# Autodesk Inventor assembly: Assembly1
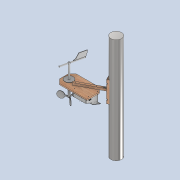
[picture p0: Inventor's stored thumbnail of the model, 180x180]
Saved by Autodesk Inventor 2022 (Build 260153000, 153)
## iProperties
Created: 2025-07-11
Part Number: Assembly1
Document SubType Name: Assembly
Designer: 1234
Author: 1234
## Documents named in this file (23)
- C:\Users\1234\Dropbox\Giorgio_Mac\PPS (pascon piccone sacchiero)\componenti\spot\IPT\Assembly1.iam
- C:\Users\1234\Dropbox\Giorgio_Mac\PPS (pascon piccone sacchiero)\componenti\spot\IPT\pannello solare.ipt
- C:\Users\1234\Dropbox\Giorgio_Mac\PPS (pascon piccone sacchiero)\componenti\spot\IPT\scatola - coperchio principale.ipt
- C:\Users\1234\Dropbox\Giorgio_Mac\PPS (pascon piccone sacchiero)\componenti\spot\IPT\Tower Pro MG996R.ipt
- C:\Users\1234\Dropbox\Giorgio_Mac\PPS (pascon piccone sacchiero)\componenti\spot\IPT\guarnizione motore.ipt
- C:\Users\1234\Dropbox\Giorgio_Mac\PPS (pascon piccone sacchiero)\componenti\spot\IPT\adattatore per motore.ipt
- C:\Users\1234\Dropbox\Giorgio_Mac\PPS (pascon piccone sacchiero)\componenti\spot\IPT\cupola alta di protezione.ipt
- C:\Users\1234\Dropbox\Giorgio_Mac\PPS (pascon piccone sacchiero)\componenti\spot\IPT\manometro.ipt
- C:\Users\1234\Dropbox\Giorgio_Mac\PPS (pascon piccone sacchiero)\componenti\spot\IPT\legno.ipt
- C:\Users\1234\Dropbox\Giorgio_Mac\PPS (pascon piccone sacchiero)\componenti\spot\IPT\direzione del vento.ipt
- C:\Users\1234\Dropbox\Giorgio_Mac\PPS (pascon piccone sacchiero)\componenti\spot\IPT\legno 1.ipt
- C:\Users\1234\Dropbox\Giorgio_Mac\PPS (pascon piccone sacchiero)\componenti\spot\IPT\legno 2.ipt
- C:\Users\1234\Dropbox\Giorgio_Mac\PPS (pascon piccone sacchiero)\componenti\spot\IPT\profiletto a l.ipt
- C:\Users\1234\Dropbox\Giorgio_Mac\PPS (pascon piccone sacchiero)\componenti\spot\IPT\lampione.ipt
- C:\Users\1234\Dropbox\Giorgio_Mac\PPS (pascon piccone sacchiero)\componenti\spot\IPT\spazzola - asta.ipt
- C:\Users\1234\Dropbox\Giorgio_Mac\PPS (pascon piccone sacchiero)\componenti\spot\IPT\spazzola - spazzola.ipt
- C:\Users\1234\Dropbox\Giorgio_Mac\PPS (pascon piccone sacchiero)\componenti\spot\IPT\spessori.ipt
- C:\Users\1234\Dropbox\Giorgio_Mac\PPS (pascon piccone sacchiero)\componenti\spot\IPT\piedino.ipt
- C:\Users\1234\Dropbox\Giorgio_Mac\PPS (pascon piccone sacchiero)\componenti\spot\IPT\tappino tpu.ipt
- C:\Users\1234\Dropbox\Giorgio_Mac\PPS (pascon piccone sacchiero)\componenti\spot\IPT\scatola - corpo - v2.ipt
- C:\Users\1234\Dropbox\Giorgio_Mac\PPS (pascon piccone sacchiero)\componenti\spot\IPT\spazzola - appoggio.ipt
- C:\Users\1234\Dropbox\Giorgio_Mac\PPS (pascon piccone sacchiero)\PCB\PCB_v2\3D_Sensor_Module_Rev_0_2025-09-11.iam
- C:\Users\1234\Dropbox\Giorgio_Mac\PPS (pascon piccone sacchiero)\componenti\spot\IPT\scatola - corpo - v3.ipt
## Components (28 placed, 22 different names)
1. scatola - coperchio principale:1 — Mate:47, Mate:49, Mate:86, Mate:109, Mate:110, Mate:134, Mate:138, Angle:3, Mate:139, Mate:145, Mate:146, Mate:147
2. pannello solare:2 — Mate:152, Angle:6
3. Tower Pro MG996R:1 — Mate:35, Mate:36, Mate:123, Mate:143, Mate:144
4. guarnizione motore:2 — Mate:125, Mate:126, Mate:127
5. adattatore per motore:2 — Mate:35, Mate:36, Mate:106, Mate:107, Mate:108
6. cupola alta di protezione:1 — Mate:140, Mate:141, Mate:142
7. legno:1 — Mate:47, Mate:49, Mate:50, Mate:54, Flush:1, Flush:2, Mate:55, Mate:56, Mate:57, Mate:64, Mate:66, Mate:78, Mate:79, Mate:80, Mate:81, Mate:82, Mate:83, Mate:84, Mate:85
8. manometro:1 — Mate:50, Mate:66, Mate:67
9. direzione del vento:1 — Mate:64, Mate:67
10. legno 1:1 — Mate:55, Mate:56, Mate:57, Mate:62, Mate:63, Flush:3, Flush:4, Mate:87, Mate:88
11. legno 2:1 — Mate:87, Mate:88, Mate:89, Mate:90, Angle:2, Mate:91
12. profiletto a l:1 — Mate:62, Flush:4, Mate:90
13. profiletto a l:2 — Mate:63, Flush:3, Mate:89
14. lampione:1 — Angle:1, Angle:2, Mate:91
15. spazzola - asta:1 — Mate:76, Flush:6, Mate:106, Mate:107, Mate:108, Mate:130
16. spazzola - spazzola:1 — Mate:76, Flush:6, Mate:130
17. spessori:1 — Mate:82, Mate:83
18. spessori:2 — Mate:81, Mate:84
19. spessori:3 — Mate:80, Mate:85, Mate:86
20. spessori:4 — Mate:78, Mate:79
21. piedino:3
22. tappino tpu:1 — Mate:148, Mate:149, Mate:150
23. scatola - corpo - v2:1 — Mate:109, Mate:110, Mate:113, Mate:123, Mate:125, Mate:126, Mate:127, Mate:131, Mate:132, Mate:134, Mate:140, Mate:141, Mate:142, Mate:143, Mate:144
24. spazzola - appoggio:1 — Mate:113, Mate:131, Mate:132
25. 3D_Sensor_Module_Rev_0_2025-09-11:1 [sub-assembly] — Mate:138, Angle:3, Mate:139
26. pannello solare:3 — Mate:151, Angle:4
27. scatola - corpo - v3:1 — Mate:145, Mate:146, Mate:147, Mate:148, Mate:149, Mate:150, Mate:151, Mate:152, Mate:153, Angle:4, Angle:5, Angle:6
28. pannello solare:4 — Mate:153, Angle:5
## Relationships (70: Mate 59, Angle 6, Flush 5)
- Mate:35: Tower Pro MG996R:1 ↔ adattatore per motore:2
- Mate:36 (0.5 mm): Tower Pro MG996R:1 ↔ adattatore per motore:2
- Mate:47: scatola - coperchio principale:1 ↔ legno:1
- Mate:49: scatola - coperchio principale:1 ↔ legno:1
- Mate:50: legno:1 ↔ manometro:1
- Mate:54: legno:1
- Flush:1: legno:1
- Flush:2: legno:1
- Mate:55: legno:1 ↔ legno 1:1
- Mate:56: legno:1 ↔ legno 1:1
- Mate:57: legno:1 ↔ legno 1:1
- Mate:62: legno 1:1 ↔ profiletto a l:1
- Mate:63: legno 1:1 ↔ profiletto a l:2
- Flush:3 (5 mm): legno 1:1 ↔ profiletto a l:2
- Flush:4 (5 mm): legno 1:1 ↔ profiletto a l:1
- Mate:64: legno:1 ↔ direzione del vento:1
- Mate:66: legno:1 ↔ manometro:1
- Mate:67: manometro:1 ↔ direzione del vento:1
- Mate:76 (0.1 mm): spazzola - asta:1 ↔ spazzola - spazzola:1
- Flush:6: spazzola - asta:1 ↔ spazzola - spazzola:1
- Mate:78: legno:1 ↔ spessori:4
- Mate:79: legno:1 ↔ spessori:4
- Mate:80: legno:1 ↔ spessori:3
- Mate:81: legno:1 ↔ spessori:2
- Mate:82: legno:1 ↔ spessori:1
- Mate:83: legno:1 ↔ spessori:1
- Mate:84: legno:1 ↔ spessori:2
- Mate:85: legno:1 ↔ spessori:3
- Mate:86: scatola - coperchio principale:1 ↔ spessori:3
- Mate:87: legno 1:1 ↔ legno 2:1
- Mate:88: legno 1:1 ↔ legno 2:1
- Mate:89: legno 2:1 ↔ profiletto a l:2
- Mate:90: legno 2:1 ↔ profiletto a l:1
- Angle:1 (0 deg): lampione:1
- Angle:2 (0 deg): legno 2:1 ↔ lampione:1
- Mate:91: legno 2:1 ↔ lampione:1
- Mate:106: adattatore per motore:2 ↔ spazzola - asta:1
- Mate:107: adattatore per motore:2 ↔ spazzola - asta:1
- Mate:108: adattatore per motore:2 ↔ spazzola - asta:1
- Mate:109: scatola - coperchio principale:1 ↔ scatola - corpo - v2:1
- Mate:110: scatola - coperchio principale:1 ↔ scatola - corpo - v2:1
- Mate:113: scatola - corpo - v2:1 ↔ spazzola - appoggio:1
- Mate:123: Tower Pro MG996R:1 ↔ scatola - corpo - v2:1
- Mate:125: guarnizione motore:2 ↔ scatola - corpo - v2:1
- Mate:126: guarnizione motore:2 ↔ scatola - corpo - v2:1
- Mate:127: guarnizione motore:2 ↔ scatola - corpo - v2:1
- Mate:130: spazzola - asta:1 ↔ spazzola - spazzola:1
- Mate:131: scatola - corpo - v2:1 ↔ spazzola - appoggio:1
- Mate:132: scatola - corpo - v2:1 ↔ spazzola - appoggio:1
- Mate:134: scatola - coperchio principale:1 ↔ scatola - corpo - v2:1
- Mate:138: scatola - coperchio principale:1 ↔ 3D_Sensor_Module_Rev_0_2025-09-11:1
- Angle:3 (0 deg): scatola - coperchio principale:1 ↔ 3D_Sensor_Module_Rev_0_2025-09-11:1
- Mate:139 (7 mm): scatola - coperchio principale:1 ↔ 3D_Sensor_Module_Rev_0_2025-09-11:1
- Mate:140: cupola alta di protezione:1 ↔ scatola - corpo - v2:1
- Mate:141: cupola alta di protezione:1 ↔ scatola - corpo - v2:1
- Mate:142: cupola alta di protezione:1 ↔ scatola - corpo - v2:1
- Mate:143: Tower Pro MG996R:1 ↔ scatola - corpo - v2:1
- Mate:144: Tower Pro MG996R:1 ↔ scatola - corpo - v2:1
- Mate:145: scatola - coperchio principale:1 ↔ scatola - corpo - v3:1
- Mate:146: scatola - coperchio principale:1 ↔ scatola - corpo - v3:1
- Mate:147: scatola - coperchio principale:1 ↔ scatola - corpo - v3:1
- Mate:148: tappino tpu:1 ↔ scatola - corpo - v3:1
- Mate:149: tappino tpu:1 ↔ scatola - corpo - v3:1
- Mate:150: tappino tpu:1 ↔ scatola - corpo - v3:1
- Mate:151: pannello solare:3 ↔ scatola - corpo - v3:1
- Mate:152: pannello solare:2 ↔ scatola - corpo - v3:1
- Mate:153: scatola - corpo - v3:1 ↔ pannello solare:4
- Angle:4 (90 deg): pannello solare:3 ↔ scatola - corpo - v3:1
- Angle:5 (0 deg): scatola - corpo - v3:1 ↔ pannello solare:4
- Angle:6 (0 deg): pannello solare:2 ↔ scatola - corpo - v3:1
